# Autodesk Inventor assembly: MotorWithPropeller
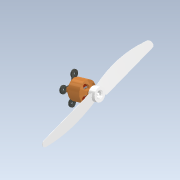
[picture p0: Inventor's stored thumbnail of the model, 180x180]
Saved by Autodesk Inventor 2021.1 (Build 251245010, 245A)
## iProperties
Created: 2024-03-20
Part Number: MotorWithPropeller
Document SubType Name: Assembly
Designer: user
Mass: 68 g
Surface Area: 259.514 cm^2
Volume: 11.4227 cm^3
Density: 5.95306 g/cm^3
Author: user
## Documents named in this file (4)
- F:\College\Semester_10\GP2\2DOF\2DOF_Hover\CAD\Workspaces\Workspace\MotorWithPropeller.iam
- F:\College\Semester_10\GP2\2DOF\2DOF_Hover\CAD\Workspaces\Workspace\Part1.ipt
- F:\College\Semester_10\GP2\2DOF\2DOF_Hover\CAD\Workspaces\Workspace\Part18.ipt
- F:\College\Semester_10\GP2\2DOF\2DOF_Hover\CAD\Workspaces\Workspace\9. Fan.ipt
## Components (3 placed, 3 different names)
1. Part1:1
2. Part18:1
3. 9. Fan:1
## Relationships (5: Mate 5)
- [Mate]: Part1:1 ↔ Part18:1
- [Mate]: Part1:1 ↔ Part18:1
- [Mate]: Part1:1 ↔ Part18:1
- [Mate]: Part1:1 ↔ 9. Fan:1
- [Mate] (5 mm): Part1:1 ↔ 9. Fan:1
